# Autodesk Inventor assembly: デフォルト指アセンブリ
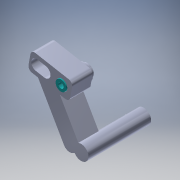
[picture p0: Inventor's stored thumbnail of the model, 180x180]
Saved by Autodesk Inventor 2018 (Build 220112000, 112)
## iProperties
Created: 2018-12-25
Part Number: デフォルト指アセンブリ
Material: 一般
Document SubType Name: Assembly
Designer: lowyu
Author: lowyu
## Documents named in this file (5)
- C:\Users\lowyu\Desktop\HAND\シャッターハンド\卒論\デフォルト指アセンブリ.iam
- C:\Users\lowyu\Desktop\HAND\シャッターハンド\指v5.ipt
- C:\Users\lowyu\Desktop\HAND\シャッターハンド\座金.ipt
- C:\Users\lowyu\Desktop\HAND\シャッターハンド\CBSA3-5 極低頭六角穴付ボルト.ipt
- C:\Users\lowyu\Desktop\HAND\シャッターハンド\内側　支柱.ipt
## Components (4 placed, 4 different names)
1. 指v5:1 — メイト:1, フラッシュ:1, メイト:2
2. 座金:1 — メイト:2, メイト:3, メイト:4, メイト:5
3. CBSA3-5 極低頭六角穴付ボルト:1 — メイト:4, メイト:5
4. 内側　支柱:2 — メイト:1, フラッシュ:1, メイト:3
## Relationships (6: Mate 5, Flush 1)
- メイト:1 [Mate]: 指v5:1 ↔ 内側　支柱:2
- フラッシュ:1 [Flush]: 指v5:1 ↔ 内側　支柱:2
- メイト:2 [Mate]: 指v5:1 ↔ 座金:1
- メイト:3 [Mate]: 座金:1 ↔ 内側　支柱:2
- メイト:4 [Mate]: 座金:1 ↔ CBSA3-5 極低頭六角穴付ボルト:1
- メイト:5 [Mate]: 座金:1 ↔ CBSA3-5 極低頭六角穴付ボルト:1
